# Autodesk Inventor assembly: ejemplo
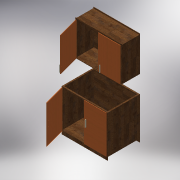
[picture p0: Inventor's stored thumbnail of the model, 180x180]
Saved by Autodesk Inventor 2016 (Build 200138000, 138)
## iProperties
Created: 2015-11-25
Part Number: ejemplo
Document SubType Name: Assembly
Designer: Daniela
Author: Daniela
## Documents named in this file (4)
- C:\Users\eolun\Desktop\Computacion\Cocina\ejemplo.iam
- C:\Users\eolun\Desktop\Computacion\Cocina\esqueleto.ipt
- C:\Users\eolun\Desktop\Computacion\Cocina\pared.ipt
- C:\Users\eolun\Desktop\Computacion\Cocina\puertas.iam
## Components (4 placed, 3 different names)
1. esqueleto:1 — Mate:3, Mate:4, Coincidencia:5, Coincidencia:6, Coincidencia:7, Nivelación:1
2. pared:1 — Coincidencia:5, Coincidencia:6, Coincidencia:8
3. pared:2 — Mate:3, Mate:4
4. puertas:1 [sub-assembly] — Coincidencia:7, Nivelación:1, Coincidencia:8
## Relationships (7: Mate 6, Flush 1)
- Mate:3: esqueleto:1 ↔ pared:2
- Mate:4: esqueleto:1 ↔ pared:2
- Coincidencia:5 [Mate]: esqueleto:1 ↔ pared:1
- Coincidencia:6 [Mate]: esqueleto:1 ↔ pared:1
- Coincidencia:7 [Mate]: esqueleto:1 ↔ puertas:1
- Nivelación:1 [Flush] (70 mm): esqueleto:1 ↔ puertas:1
- Coincidencia:8 [Mate] (10 mm): pared:1 ↔ puertas:1
